# Autodesk Inventor assembly: アーム 2段目ギアアセンブリ 8 64.ipt
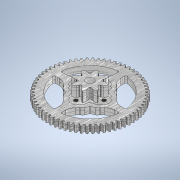
[picture p0: Inventor's stored thumbnail of the model, 180x180]
Saved by Autodesk Inventor 2020.2 (Build 242310000, 310)
## iProperties
Created: 2020-05-01
Part Number: アーム 2段目ギアアセンブリ 8 64.ipt
Document SubType Name: Assembly
Designer: mozar
Author: mozar
## Documents named in this file (4)
- C:\Users\mozar\Desktop\院2年機大型\アーム 2段目ギアアセンブリ 8 64.ipt.iam
- C:\Users\mozar\Desktop\院2年機大型\アーム 2段目ギア 大ギア 64.ipt
- C:\Users\mozar\Desktop\院2年機大型\アーム 2段目ギア 小ギア 8.ipt
- C:\Users\mozar\Desktop\院2年機大型\既製品\ねじ\SB　5mm皿ネジ.ipt
## Components (6 placed, 3 different names)
1. アーム 2段目ギア 大ギア 64:1 — 挿入:1, 挿入:2, 挿入:3, 挿入:4, 挿入:5, 挿入:6
2. アーム 2段目ギア 小ギア 8:1 — 挿入:1, 挿入:2
3. SB　5mm皿ネジ:1 — 挿入:3
4. SB　5mm皿ネジ:2 — 挿入:4
5. SB　5mm皿ネジ:3 — 挿入:6
6. SB　5mm皿ネジ:4 — 挿入:5
## Relationships (6: Insert 6)
- 挿入:1 [Insert]: アーム 2段目ギア 大ギア 64:1 ↔ アーム 2段目ギア 小ギア 8:1
- 挿入:2 [Insert]: アーム 2段目ギア 大ギア 64:1 ↔ アーム 2段目ギア 小ギア 8:1
- 挿入:3 [Insert]: アーム 2段目ギア 大ギア 64:1 ↔ SB　5mm皿ネジ:1
- 挿入:4 [Insert]: アーム 2段目ギア 大ギア 64:1 ↔ SB　5mm皿ネジ:2
- 挿入:5 [Insert]: アーム 2段目ギア 大ギア 64:1 ↔ SB　5mm皿ネジ:4
- 挿入:6 [Insert]: アーム 2段目ギア 大ギア 64:1 ↔ SB　5mm皿ネジ:3
